# Autodesk Inventor assembly: ChassisBase
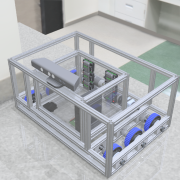
[picture p0: Inventor's stored thumbnail of the model, 180x180]
Saved by Autodesk Inventor 2018 (Build 220112000, 112)
## iProperties
Created: 2017-09-03
Part Number: ChassisBase
Document SubType Name: Assembly
Designer: snipe
Mass: 4555.63 g
Surface Area: 31405.8 cm^2
Volume: 4555.63 cm^3
Density: 1 g/cm^3
Author: snipe
## Documents named in this file (15)
- C:\Users\snipe\Documents\Clark\CAD Assets\ClarkBodyV3.iam
- C:\Users\snipe\Documents\Clark\CAD Assets\pro20in.ipt
- C:\Users\snipe\Documents\Clark\CAD Assets\DriveShaftA.iam
- C:\Users\snipe\Documents\Clark\CAD Assets\SideShaftA.iam
- C:\Users\snipe\Documents\Clark\CAD Assets\SideShaftB.iam
- C:\Users\snipe\Documents\Clark\CAD Assets\Profile_BaseModel_20mm\Profile_BaseModel_20mm-02.ipt
- E:\Clark\Assets\Profile_BaseModel_20mm.ipt
- C:\Users\snipe\Documents\Clark\CAD Assets\VPlan775dualinput.iam
- C:\Users\snipe\Documents\Clark\CAD Assets\24tPulley15mm.ipt
- C:\Users\snipe\Documents\Clark\CAD Assets\ShaftCollar.ipt
- C:\Users\snipe\Documents\Clark\CAD Assets\Profile_BaseModel_20mm\Profile_BaseModel_20mm-10.ipt
- C:\Users\snipe\Documents\Clark\CAD Assets\5.5belt.ipt
- C:\Users\snipe\Documents\Clark\CAD Assets\Profile_BaseModel_20mm\Profile_BaseModel_20mm-13.ipt
- C:\Users\snipe\Documents\Clark\CAD Assets\BrainBoxV1.iam
- C:\Users\snipe\Documents\Clark\CAD Assets\BearingBlock30mmRight.ipt
## Components (52 placed, 24 different names)
1. 5.5belt:1 — Mate:197
2. BrainBoxV1:1 [sub-assembly] — Mate:202, Mate:203, Flush:224
3. Profile_BaseModel_20mm-10:23 — Mate:184, Flush:190, Flush:191, Mate:187, Flush:200, Flush:201, Mate:194
4. Profile_BaseModel_20mm-10:26 — Mate:188, Flush:202, Flush:203, Mate:191
5. pro20in:1 — Mate:31, Flush:19, Mate:32, Mate:33, Flush:20, Flush:21, Mate:128, Flush:110, Flush:111, Mate:129, Flush:112, Flush:113, Flush:211
6. pro20in:2 — Mate:9, Flush:9, Mate:11, Flush:10, Flush:11, Mate:20, Flush:15, Mate:125, Flush:104, Flush:105, Flush:118, Mate:132, Flush:119, Flush:203
7. pro20in:3 — Flush:16, Mate:28, Flush:17, Mate:29, Flush:18, Mate:30, Flush:201, Mate:191, Flush:208
8. pro20in:4 — Mate:15, Mate:16, Flush:12, Flush:13, Flush:14, Mate:19, Flush:15, Flush:200, Mate:194, Flush:210
9. SideShaftA:1 [sub-assembly] — Mate:21, Mate:22, Mate:27, Mate:145, Mate:147, Mate:149
10. DriveShaftA:1 [sub-assembly] — Mate:23, Mate:24, Mate:140, Mate:147, Mate:148, Flush:149, Mate:173, Flush:184
11. SideShaftB:1 [sub-assembly] — Mate:25, Mate:26, Mate:141, Mate:148
12. SideShaftB:2 [sub-assembly] — Mate:88, Mate:93, Mate:144, Mate:149
13. DriveShaftA:2 [sub-assembly] — Mate:85, Mate:92, Mate:139, Mate:146, Flush:149, Mate:172, Flush:185
14. SideShaftA:2 [sub-assembly] — Mate:86, Mate:87, Mate:90, Mate:91, Mate:146
15. RightBack — Mate:11, Flush:11, Mate:141, Flush:143
16. RightCenter — Flush:10, Mate:20, Mate:140, Flush:144
17. RightFront — Mate:9, Flush:9, Mate:27, Mate:145, Flush:145, Mate:157
18. RightBack2 — Mate:16, Flush:14, Mate:17, Mate:25, Mate:26, Flush:141, Flush:143
19. RightCenter2 — Flush:12, Mate:17, Mate:18, Mate:19, Mate:23, Mate:24, Flush:140, Flush:144
20. RightFront2 — Mate:15, Flush:13, Mate:18, Mate:21, Mate:22, Flush:139, Flush:142, Flush:145, Mate:156
21. LeftBack — Mate:32, Flush:21, Mate:86, Mate:87, Mate:89, Flush:148
22. LeftCenter — Mate:31, Flush:19, Mate:35, Mate:85, Mate:89, Mate:92, Flush:147, Flush:211
23. LeftFront — Mate:33, Flush:20, Mate:35, Mate:88, Mate:93, Flush:146
24. LeftBack2 — Flush:18, Mate:30, Mate:90, Mate:91, Flush:141, Flush:148
25. LeftCenter2 — Flush:17, Mate:29, Mate:139, Flush:140, Flush:147
26. LeftFront2 — Flush:16, Mate:28, Flush:139, Mate:144, Flush:142, Flush:146
27. Profile_BaseModel_20mm-10:24 — Mate:185, Flush:194, Flush:195, Flush:196, Flush:197, Flush:198, Flush:199, Mate:195, Mate:196, Mate:198, Mate:199, Flush:213, Flush:215
28. Profile_BaseModel_20mm-10:27 — Mate:189, Flush:204, Flush:205, Mate:192, Mate:193, Flush:209, Mate:200, Mate:201, Flush:217, Flush:218
29. pro20in:9 — Flush:173, Mate:169, Flush:176, Mate:170, Flush:196, Mate:192
30. pro20in:10 — Mate:168, Flush:175, Mate:171, Flush:199, Mate:196, Mate:203, Flush:224
31. pro20in:5 — Mate:150, Flush:153, Mate:157, Flush:204
32. pro20in:6 — Mate:156, Mate:171, Flush:198, Flush:210, Mate:195, Flush:222, Flush:223
33. pro20in:7 — Flush:173, Mate:170, Flush:197, Flush:208, Mate:193, Flush:220, Flush:221
34. pro20in:8 — Mate:153, Flush:150, Flush:194
35. Profile_BaseModel_20mm-13:29 — Mate:198, Flush:213, Flush:220
36. Profile_BaseModel_20mm-13:30 — Mate:199, Flush:215, Flush:223
37. Profile_BaseModel_20mm-13:31 — Mate:200, Flush:217, Flush:221
38. Profile_BaseModel_20mm-13:32 — Mate:201, Flush:218, Flush:222
39. Profile_BaseModel_20mm-02:1 — Mate:125, Flush:104, Flush:105, Mate:138, Flush:133, Flush:134, Mate:182, Mate:183, Mate:187
40. Profile_BaseModel_20mm-02:4 — Mate:128, Flush:110, Flush:111, Mate:184, Flush:190, Flush:191, Mate:185, Mate:186, Flush:192, Flush:193, Flush:195
41. Profile_BaseModel_20mm-02:5 — Mate:129, Flush:112, Flush:113, Mate:153, Flush:150, Mate:180, Flush:186, Flush:187, Mate:188, Mate:189, Mate:190, Flush:209
42. Profile_BaseModel_20mm-02:8 — Flush:118, Mate:132, Flush:119, Mate:150, Flush:153, Mate:181, Flush:188, Flush:189, Flush:202, Flush:205, Flush:206
43. Profile_BaseModel_20mm-10:25 — Mate:186, Flush:192, Flush:193, Mate:202
44. Profile_BaseModel_20mm-10:28 — Mate:190, Flush:206, Flush:207
45. pro20in:11 — Mate:180, Flush:186, Flush:187
46. pro20in:12 — Mate:181, Flush:188, Flush:189, Mate:182, Mate:183, Flush:207
47. VPlan775dualinput:1 [sub-assembly] — Mate:169, Flush:176, Mate:172, Mate:178, Mate:179
48. VPlan775dualinput:2 [sub-assembly] — Mate:168, Flush:175, Mate:173, Mate:176, Mate:177
49. 24tPulley15mm:1 — Flush:177, Flush:178, Mate:176, Mate:177, Flush:184, Mate:197
50. ShaftCollar:1 — Flush:177, Flush:178
51. 24tPulley15mm:2 — Flush:182, Flush:183, Mate:178, Mate:179, Flush:185
52. ShaftCollar:2 — Flush:182, Flush:183
## Relationships (165: Mate 85, Flush 80)
- Mate:9: pro20in:2 ↔ RightFront
- Flush:9: pro20in:2 ↔ RightFront
- Mate:11: pro20in:2 ↔ RightBack
- Flush:10: pro20in:2 ↔ RightCenter
- Flush:11: pro20in:2 ↔ RightBack
- Mate:15: pro20in:4 ↔ RightFront2
- Mate:16: pro20in:4 ↔ RightBack2
- Flush:12: pro20in:4 ↔ RightCenter2
- Flush:13: pro20in:4 ↔ RightFront2
- Flush:14: pro20in:4 ↔ RightBack2
- Mate:17 (-147.447 mm): RightBack2 ↔ RightCenter2
- Mate:18 (147.447 mm): RightCenter2 ↔ RightFront2
- Mate:19: pro20in:4 ↔ RightCenter2
- Mate:20: pro20in:2 ↔ RightCenter
- Mate:21: SideShaftA:1 ↔ RightFront2
- Mate:22: SideShaftA:1 ↔ RightFront2
- Mate:23: DriveShaftA:1 ↔ RightCenter2
- Mate:24: DriveShaftA:1 ↔ RightCenter2
- Mate:25: SideShaftB:1 ↔ RightBack2
- Mate:26: SideShaftB:1 ↔ RightBack2
- Mate:27: SideShaftA:1 ↔ RightFront
- Flush:15: pro20in:2 ↔ pro20in:4
- Flush:16: pro20in:3 ↔ LeftFront2
- Mate:28: pro20in:3 ↔ LeftFront2
- Flush:17: pro20in:3 ↔ LeftCenter2
- Mate:29: pro20in:3 ↔ LeftCenter2
- Flush:18: pro20in:3 ↔ LeftBack2
- Mate:30: pro20in:3 ↔ LeftBack2
- Mate:31: pro20in:1 ↔ LeftCenter
- Flush:19: pro20in:1 ↔ LeftCenter
- Mate:32: pro20in:1 ↔ LeftBack
- Mate:33: pro20in:1 ↔ LeftFront
- Flush:20: pro20in:1 ↔ LeftFront
- Flush:21: pro20in:1 ↔ LeftBack
- Mate:35 (147.447 mm): LeftCenter ↔ LeftFront
- Mate:85: DriveShaftA:2 ↔ LeftCenter
- Mate:86: SideShaftA:2 ↔ LeftBack
- Mate:87: SideShaftA:2 ↔ LeftBack
- Mate:88: SideShaftB:2 ↔ LeftFront
- Mate:89 (147.447 mm): LeftBack ↔ LeftCenter
- Mate:90: SideShaftA:2 ↔ LeftBack2
- Mate:91: SideShaftA:2 ↔ LeftBack2
- Mate:92: DriveShaftA:2 ↔ LeftCenter
- Mate:93: SideShaftB:2 ↔ LeftFront
- Mate:125: pro20in:2 ↔ Profile_BaseModel_20mm-02:1
- Flush:104: pro20in:2 ↔ Profile_BaseModel_20mm-02:1
- Flush:105: pro20in:2 ↔ Profile_BaseModel_20mm-02:1
- Mate:128: pro20in:1 ↔ Profile_BaseModel_20mm-02:4
- Flush:110: pro20in:1 ↔ Profile_BaseModel_20mm-02:4
- Flush:111: pro20in:1 ↔ Profile_BaseModel_20mm-02:4
- Mate:129: pro20in:1 ↔ Profile_BaseModel_20mm-02:5
- Flush:112: pro20in:1 ↔ Profile_BaseModel_20mm-02:5
- Flush:113: pro20in:1 ↔ Profile_BaseModel_20mm-02:5
- Flush:118: pro20in:2 ↔ Profile_BaseModel_20mm-02:8
- Mate:132: pro20in:2 ↔ Profile_BaseModel_20mm-02:8
- Flush:119: pro20in:2 ↔ Profile_BaseModel_20mm-02:8
- Mate:138: Profile_BaseModel_20mm-02:1
- Flush:133: Profile_BaseModel_20mm-02:1
- Flush:134: Profile_BaseModel_20mm-02:1
- Mate:139: DriveShaftA:2 ↔ LeftCenter2
- Mate:140: DriveShaftA:1 ↔ RightCenter
- Mate:141: SideShaftB:1 ↔ RightBack
- Flush:139: RightFront2 ↔ LeftFront2
- Mate:144: SideShaftB:2 ↔ LeftFront2
- Mate:145: SideShaftA:1 ↔ RightFront
- Flush:140: RightCenter2 ↔ LeftCenter2
- Flush:141: RightBack2 ↔ LeftBack2
- Flush:142: RightFront2 ↔ LeftFront2
- Flush:143: RightBack ↔ RightBack2
- Flush:144: RightCenter ↔ RightCenter2
- Flush:145: RightFront ↔ RightFront2
- Flush:146: LeftFront ↔ LeftFront2
- Flush:147: LeftCenter ↔ LeftCenter2
- Flush:148: LeftBack ↔ LeftBack2
- Mate:146: DriveShaftA:2 ↔ SideShaftA:2
- Mate:147: SideShaftA:1 ↔ DriveShaftA:1
- Mate:148: DriveShaftA:1 ↔ SideShaftB:1
- Flush:149: DriveShaftA:1 ↔ DriveShaftA:2
- Mate:149: SideShaftA:1 ↔ SideShaftB:2
- Mate:150: pro20in:5 ↔ Profile_BaseModel_20mm-02:8
- Mate:153: pro20in:8 ↔ Profile_BaseModel_20mm-02:5
- Flush:150: pro20in:8 ↔ Profile_BaseModel_20mm-02:5
- Flush:153: pro20in:5 ↔ Profile_BaseModel_20mm-02:8
- Mate:156: RightFront2 ↔ pro20in:6
- Mate:157: RightFront ↔ pro20in:5
- Flush:173: pro20in:9 ↔ pro20in:7
- Mate:168: pro20in:10 ↔ VPlan775dualinput:2
- Flush:175: pro20in:10 ↔ VPlan775dualinput:2
- Mate:169: pro20in:9 ↔ VPlan775dualinput:1
- Flush:176: pro20in:9 ↔ VPlan775dualinput:1
- Mate:170 (26.9875 mm): pro20in:9 ↔ pro20in:7
- Mate:171 (26.9875 mm): pro20in:10 ↔ pro20in:6
- Mate:172 (140.0251 mm): DriveShaftA:2 ↔ VPlan775dualinput:1
- Mate:173 (140.0251 mm): DriveShaftA:1 ↔ VPlan775dualinput:2
- [Mate]: 24tPulley15mm:1 ↔ ShaftCollar:1
- [Mate]: 24tPulley15mm:2 ↔ ShaftCollar:2
- Flush:177: 24tPulley15mm:1 ↔ ShaftCollar:1
- Flush:178: 24tPulley15mm:1 ↔ ShaftCollar:1
- Mate:176: VPlan775dualinput:2 ↔ 24tPulley15mm:1
- Mate:177: VPlan775dualinput:2 ↔ 24tPulley15mm:1
- Flush:182: 24tPulley15mm:2 ↔ ShaftCollar:2
- Flush:183: 24tPulley15mm:2 ↔ ShaftCollar:2
- Mate:178: VPlan775dualinput:1 ↔ 24tPulley15mm:2
- Mate:179: VPlan775dualinput:1 ↔ 24tPulley15mm:2
- Flush:184: DriveShaftA:1 ↔ 24tPulley15mm:1
- Flush:185: DriveShaftA:2 ↔ 24tPulley15mm:2
- Mate:180: Profile_BaseModel_20mm-02:5 ↔ pro20in:11
- Flush:186: Profile_BaseModel_20mm-02:5 ↔ pro20in:11
- Flush:187: Profile_BaseModel_20mm-02:5 ↔ pro20in:11
- Mate:181: Profile_BaseModel_20mm-02:8 ↔ pro20in:12
- Flush:188: Profile_BaseModel_20mm-02:8 ↔ pro20in:12
- Flush:189: Profile_BaseModel_20mm-02:8 ↔ pro20in:12
- Mate:182: Profile_BaseModel_20mm-02:1 ↔ pro20in:12
- Mate:183: Profile_BaseModel_20mm-02:1 ↔ pro20in:12
- Mate:184: Profile_BaseModel_20mm-10:23 ↔ Profile_BaseModel_20mm-02:4
- Flush:190: Profile_BaseModel_20mm-10:23 ↔ Profile_BaseModel_20mm-02:4
- Flush:191: Profile_BaseModel_20mm-10:23 ↔ Profile_BaseModel_20mm-02:4
- Mate:185: Profile_BaseModel_20mm-10:24 ↔ Profile_BaseModel_20mm-02:4
- Mate:186: Profile_BaseModel_20mm-02:4 ↔ Profile_BaseModel_20mm-10:25
- Flush:192: Profile_BaseModel_20mm-02:4 ↔ Profile_BaseModel_20mm-10:25
- Flush:193: Profile_BaseModel_20mm-02:4 ↔ Profile_BaseModel_20mm-10:25
- Flush:194: Profile_BaseModel_20mm-10:24 ↔ pro20in:8
- Flush:195: Profile_BaseModel_20mm-10:24 ↔ Profile_BaseModel_20mm-02:4
- Flush:196: Profile_BaseModel_20mm-10:24 ↔ pro20in:9
- Flush:197: Profile_BaseModel_20mm-10:24 ↔ pro20in:7
- Mate:187: Profile_BaseModel_20mm-10:23 ↔ Profile_BaseModel_20mm-02:1
- Flush:198: Profile_BaseModel_20mm-10:24 ↔ pro20in:6
- Flush:199: Profile_BaseModel_20mm-10:24 ↔ pro20in:10
- Flush:200: Profile_BaseModel_20mm-10:23 ↔ pro20in:4
- Flush:201: Profile_BaseModel_20mm-10:23 ↔ pro20in:3
- Mate:188: Profile_BaseModel_20mm-10:26 ↔ Profile_BaseModel_20mm-02:5
- Mate:189: Profile_BaseModel_20mm-10:27 ↔ Profile_BaseModel_20mm-02:5
- Mate:190: Profile_BaseModel_20mm-02:5 ↔ Profile_BaseModel_20mm-10:28
- Flush:202: Profile_BaseModel_20mm-10:26 ↔ Profile_BaseModel_20mm-02:8
- Flush:203: Profile_BaseModel_20mm-10:26 ↔ pro20in:2
- Flush:204: Profile_BaseModel_20mm-10:27 ↔ pro20in:5
- Flush:205: Profile_BaseModel_20mm-10:27 ↔ Profile_BaseModel_20mm-02:8
- Flush:206: Profile_BaseModel_20mm-02:8 ↔ Profile_BaseModel_20mm-10:28
- Flush:207: Profile_BaseModel_20mm-10:28 ↔ pro20in:12
- Mate:191: Profile_BaseModel_20mm-10:26 ↔ pro20in:3
- Flush:208: pro20in:3 ↔ pro20in:7
- Mate:192: Profile_BaseModel_20mm-10:27 ↔ pro20in:9
- Mate:193: Profile_BaseModel_20mm-10:27 ↔ pro20in:7
- Flush:209: Profile_BaseModel_20mm-10:27 ↔ Profile_BaseModel_20mm-02:5
- Mate:194: Profile_BaseModel_20mm-10:23 ↔ pro20in:4
- Flush:210: pro20in:4 ↔ pro20in:6
- Mate:195: Profile_BaseModel_20mm-10:24 ↔ pro20in:6
- Mate:196: Profile_BaseModel_20mm-10:24 ↔ pro20in:10
- Flush:211: pro20in:1 ↔ LeftCenter
- Mate:197: 5.5belt:1 ↔ 24tPulley15mm:1
- Mate:198: Profile_BaseModel_20mm-10:24 ↔ Profile_BaseModel_20mm-13:29
- Mate:199: Profile_BaseModel_20mm-10:24 ↔ Profile_BaseModel_20mm-13:30
- Mate:200: Profile_BaseModel_20mm-10:27 ↔ Profile_BaseModel_20mm-13:31
- Mate:201: Profile_BaseModel_20mm-10:27 ↔ Profile_BaseModel_20mm-13:32
- Flush:213: Profile_BaseModel_20mm-10:24 ↔ Profile_BaseModel_20mm-13:29
- Flush:215: Profile_BaseModel_20mm-10:24 ↔ Profile_BaseModel_20mm-13:30
- Flush:217: Profile_BaseModel_20mm-10:27 ↔ Profile_BaseModel_20mm-13:31
- Flush:218: Profile_BaseModel_20mm-10:27 ↔ Profile_BaseModel_20mm-13:32
- Flush:220: pro20in:7 ↔ Profile_BaseModel_20mm-13:29
- Flush:221: pro20in:7 ↔ Profile_BaseModel_20mm-13:31
- Flush:222: pro20in:6 ↔ Profile_BaseModel_20mm-13:32
- Flush:223: pro20in:6 ↔ Profile_BaseModel_20mm-13:30
- Mate:202: BrainBoxV1:1 ↔ Profile_BaseModel_20mm-10:25
- Mate:203: BrainBoxV1:1 ↔ pro20in:10
- Flush:224: BrainBoxV1:1 ↔ pro20in:10
## Named parameters: d478_d283 = 0 mm, sa_0 = -5.66886e-06, sa_1 = -53378.7, sa_2 = -2.491e-11
note: some values were not read from the file. Shown as the stored number, unit unknown: "sa_0", "sa_1", "sa_2".
